# Autodesk Inventor assembly: craft
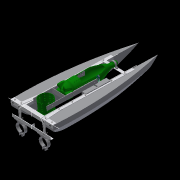
[picture p0: Inventor's stored thumbnail of the model, 180x180]
Saved by Autodesk Inventor 2016 (Build 200138000, 138)
## iProperties
Created: 2019-02-12
Part Number: craft
Document SubType Name: Assembly
Designer: Calb3e
Author: Calb3e
## Documents named in this file (24)
- C:\Users\Calb3\Documents\Inventor\water proj\craft.iam
- C:\Users\Calb3\Documents\Inventor\water proj\GeneralCraftShape4 (1).ipt
- C:\Users\Calb3\Documents\Inventor\water proj\Water Bottle.ipt
- C:\Users\Calb3\Documents\Inventor\water proj\Lbarx2.ipt
- C:\Users\Calb3\Documents\Inventor\water proj\half bottle.ipt
- C:\Users\Calb3\Documents\Inventor\water proj\Lbarx1 big.ipt
- C:\Users\Calb3\Documents\Inventor\water proj\flat bar1.ipt
- C:\Users\Calb3\Documents\Inventor\water proj\holder.ipt
- C:\Users\Calb3\Documents\Inventor\water proj\flatbarx2.ipt
- C:\Users\Calb3\Documents\Inventor\water proj\Lbarx1 small.ipt
- C:\Users\Calb3\Documents\Inventor\water proj\cushion.ipt
- C:\Users\Calb3\Documents\Inventor\water proj\pumpholder (1).ipt
- C:\Users\Calb3\Documents\Inventor\Content Center Files\R2016\en-US\ISO 7089\ISO 7089 - 5 - 140 HV(1).ipt
- C:\Users\Calb3\Documents\Inventor\Content Center Files\R2016\en-US\ISO 4762(2)\ISO 4762 - M5 x 20ISO.ipt
- C:\Users\Calb3\Documents\Inventor\Content Center Files\R2016\en-US\ISO 4032(2)\ISO 4032 - M5 - ISO.ipt
- C:\Users\Calb3\Documents\Inventor\Content Center Files\R2016\en-US\Wood screw 4 GOST 1145-80\Wood screw 4-5x22 GOST 1145-80.ipt
- C:\Users\Calb3\Documents\Inventor\Content Center Files\R2016\en-US\Screw GB_T 951-1986\Screw GB_T 951-1986 5 x 30.ipt
- C:\Users\Calb3\Documents\Inventor\water proj\extension.ipt
- C:\Users\Calb3\Documents\Inventor\water proj\extension2.ipt
- C:\Users\Calb3\Documents\Inventor\water proj\extension3.ipt
- C:\Users\Calb3\Documents\Inventor\water proj\support.ipt
- C:\Users\Calb3\Documents\Inventor\Content Center Files\R2016\en-US\ISO 4762(2)\ISO 4762 - M3 x 30ISO.ipt
- C:\Users\Calb3\Documents\Inventor\Content Center Files\R2016\en-US\ISO 4032(2)\ISO 4032 - M3 - ISO.ipt
- C:\Users\Calb3\Documents\Inventor\water proj\lastflat bar.ipt
## Components (88 placed, 23 different names)
1. GeneralCraftShape4 (1):1 — Mate:1, Mate:2, Mate:3, Mate:4, Mate:6, Angle:1
2. Lbarx2:1 — Mate:3, Mate:4, Mate:7, Insert:1, Mate:9, Mate:10, Mate:11, Mate:12, Insert:33, Insert:34, Insert:35, Insert:36
3. Lbarx2:2 — Mate:1, Mate:2, Insert:2, Mate:13, Mate:14, Mate:15, Mate:16, Insert:27, Insert:28, Insert:30, Insert:31, Insert:82
4. Water Bottle:1 — Insert:5, Angle:1
5. half bottle:1 — Mate:21
6. Lbarx1 big:1 — Mate:6, Mate:7, Insert:6, Insert:7, Insert:84
7. flat bar1:1 — Insert:1, Insert:2, Insert:3, Insert:4, Insert:29, Insert:32, Insert:50, Insert:51
8. holder:1 — Insert:3, Insert:4, Insert:5, Insert:38, Insert:39
9. flatbarx2:1 — Insert:7, Insert:9, Insert:23, Insert:24
10. flatbarx2:2 — Insert:6, Insert:8, Insert:19, Insert:20
11. Lbarx1 small:2 — Insert:8, Insert:9, Insert:10, Insert:11, Insert:12, Insert:13, Insert:21, Insert:22, Insert:42, Insert:43, Insert:44, Insert:45
12. cushion:1 — Mate:11, Mate:12
13. cushion:2 — Mate:13, Mate:14
14. cushion:3 — Mate:9, Mate:10
15. cushion:4 — Mate:15, Mate:16
16. pumpholder (1):1 — Insert:10, Insert:11, Insert:46, Insert:47
17. pumpholder (1):2 — Insert:12, Insert:13, Insert:48, Insert:49
18. ISO 7089 5 - 140 HV:1 — Insert:35, Insert:73
19. ISO 7089 5 - 140 HV:2 — Insert:32, Insert:70
20. ISO 7089 5 - 140 HV:3 — Insert:31, Insert:68
21. ISO 7089 5 - 140 HV:4 — Insert:30, Insert:67
22. ISO 7089 5 - 140 HV:5 — Insert:29, Insert:69
23. ISO 7089 5 - 140 HV:6 — Insert:28, Insert:66
24. ISO 7089 5 - 140 HV:12 — Insert:36, Insert:74
25. ISO 7089 5 - 140 HV:13 — Insert:34, Insert:72
26. ISO 7089 5 - 140 HV:14 — Insert:33, Insert:71
27. ISO 7089 5 - 140 HV:15 — Insert:59
28. ISO 7089 5 - 140 HV:18 — Insert:56
29. ISO 7089 5 - 140 HV:20 — Insert:22, Insert:62
30. ISO 7089 5 - 140 HV:21 — Insert:53
31. ISO 7089 5 - 140 HV:22 — Insert:19, Insert:52
32. ISO 7089 5 - 140 HV:23 — Insert:24, Insert:54
33. ISO 7089 5 - 140 HV:24 — Insert:23, Insert:61
34. ISO 7089 5 - 140 HV:25 — Insert:27, Insert:65
35. ISO 7089 5 - 140 HV:27 — Insert:55
36. ISO 7089 5 - 140 HV:28 — Insert:20, Insert:64
37. ISO 7089 5 - 140 HV:29 — Insert:21, Insert:63
38. ISO 4762 M5 x 20:1 — Insert:41
39. ISO 4762 M5 x 20:2 — Insert:40
40. ISO 4762 M5 x 20:3 — Insert:44
41. ISO 4762 M5 x 20:4 — Insert:45
42. ISO 4762 M5 x 20:5 — Insert:43
43. ISO 4762 M5 x 20:6 — Insert:42
44. ISO 7089 5 - 140 HV:30 — Insert:39, Insert:41
45. ISO 7089 5 - 140 HV:31 — Insert:38, Insert:40
46. ISO 4032 M5:1 — Insert:46
47. ISO 4032 M5:2 — Insert:47
48. ISO 4032 M5:3 — Insert:49
49. ISO 4032 M5:4 — Insert:48
50. ISO 4032 M5:5 — Insert:51
51. ISO 4032 M5:6 — Insert:50
52. Wood screw 4 GOST 1145-80 5x(22):1 — Insert:53
53. Wood screw 4 GOST 1145-80 5x(22):2 — Insert:55
54. Wood screw 4 GOST 1145-80 5x(22):3 — Insert:52
55. Wood screw 4 GOST 1145-80 5x(22):4 — Insert:54
56. Wood Screw GB/T 951-1986 M2.2 x 4.5-5-30:1 — Insert:61
57. Wood Screw GB/T 951-1986 M2.2 x 4.5-5-30:3 — Insert:62
58. Wood Screw GB/T 951-1986 M2.2 x 4.5-5-30:4 — Insert:63
59. Wood Screw GB/T 951-1986 M2.2 x 4.5-5-30:7 — Insert:56
60. Wood Screw GB/T 951-1986 M2.2 x 4.5-5-30:8 — Insert:59
61. Wood Screw GB/T 951-1986 M2.2 x 4.5-5-30:9 — Insert:64
62. Wood Screw GB/T 951-1986 M2.2 x 4.5-5-30:10 — Insert:65
63. Wood Screw GB/T 951-1986 M2.2 x 4.5-5-30:11 — Insert:66
64. Wood Screw GB/T 951-1986 M2.2 x 4.5-5-30:12 — Insert:68
65. Wood Screw GB/T 951-1986 M2.2 x 4.5-5-30:13 — Insert:67
66. Wood Screw GB/T 951-1986 M2.2 x 4.5-5-30:14 — Insert:69
67. Wood Screw GB/T 951-1986 M2.2 x 4.5-5-30:16 — Insert:74
68. Wood Screw GB/T 951-1986 M2.2 x 4.5-5-30:17 — Insert:73
69. Wood Screw GB/T 951-1986 M2.2 x 4.5-5-30:18 — Insert:72
70. Wood Screw GB/T 951-1986 M2.2 x 4.5-5-30:19 — Insert:71
71. Wood Screw GB/T 951-1986 M2.2 x 4.5-5-30:20 — Insert:70
72. extension:1 — Insert:76, Insert:77, Mate:18, Flush:2, Mate:19
73. extension2:1 — Insert:78, Insert:79, Mate:17, Flush:1, Mate:20, Mate:21, Insert:80
74. extension3:1 — Insert:78, Insert:79
75. extension3:2 — Insert:76, Insert:77
76. support:1 — Mate:17, Flush:1, Mate:18, Flush:2, Mate:19, Mate:20
77. ISO 4762 M3 x 30:1 — Insert:80, Mate:22, Flush:3
78. ISO 4032 M3:1 — Mate:22, Flush:3
79. lastflat bar:1 — Insert:82, Insert:87, Insert:88
80. lastflat bar:2 — Insert:84, Insert:85, Insert:86
81. Wood Screw GB/T 951-1986 M2.2 x 4.5-5-30:21 — Insert:92
82. Wood Screw GB/T 951-1986 M2.2 x 4.5-5-30:22 — Insert:89
83. Wood Screw GB/T 951-1986 M2.2 x 4.5-5-30:23 — Insert:91
84. Wood Screw GB/T 951-1986 M2.2 x 4.5-5-30:24 — Insert:90
85. ISO 7089 5 - 140 HV:32 — Insert:87, Insert:92
86. ISO 7089 5 - 140 HV:33 — Insert:86, Insert:91
87. ISO 7089 5 - 140 HV:34 — Insert:85, Insert:90
88. ISO 7089 5 - 140 HV:35 — Insert:88, Insert:89
## Relationships (102: Insert 78, Mate 20, Flush 3, Angle 1)
- Mate:1: GeneralCraftShape4 (1):1 ↔ Lbarx2:2
- Mate:2: GeneralCraftShape4 (1):1 ↔ Lbarx2:2
- Mate:3: GeneralCraftShape4 (1):1 ↔ Lbarx2:1
- Mate:4: GeneralCraftShape4 (1):1 ↔ Lbarx2:1
- Mate:6: GeneralCraftShape4 (1):1 ↔ Lbarx1 big:1
- Mate:7: Lbarx2:1 ↔ Lbarx1 big:1
- Insert:1: Lbarx2:1 ↔ flat bar1:1
- Insert:2: Lbarx2:2 ↔ flat bar1:1
- Insert:3: flat bar1:1 ↔ holder:1
- Insert:4: flat bar1:1 ↔ holder:1
- Insert:5: Water Bottle:1 ↔ holder:1
- Angle:1 (90 deg): GeneralCraftShape4 (1):1 ↔ Water Bottle:1
- Insert:6: Lbarx1 big:1 ↔ flatbarx2:2
- Insert:7: Lbarx1 big:1 ↔ flatbarx2:1
- Insert:8: flatbarx2:2 ↔ Lbarx1 small:2
- Insert:9: flatbarx2:1 ↔ Lbarx1 small:2
- Mate:9: Lbarx2:1 ↔ cushion:3
- Mate:10: Lbarx2:1 ↔ cushion:3
- Mate:11: Lbarx2:1 ↔ cushion:1
- Mate:12: Lbarx2:1 ↔ cushion:1
- Mate:13: Lbarx2:2 ↔ cushion:2
- Mate:14: Lbarx2:2 ↔ cushion:2
- Mate:15: Lbarx2:2 ↔ cushion:4
- Mate:16: Lbarx2:2 ↔ cushion:4
- Insert:10: Lbarx1 small:2 ↔ pumpholder (1):1
- Insert:11: Lbarx1 small:2 ↔ pumpholder (1):1
- Insert:12: Lbarx1 small:2 ↔ pumpholder (1):2
- Insert:13: Lbarx1 small:2 ↔ pumpholder (1):2
- Insert:19: flatbarx2:2 ↔ ISO 7089 5 - 140 HV:22
- Insert:20: flatbarx2:2 ↔ ISO 7089 5 - 140 HV:28
- Insert:21: Lbarx1 small:2 ↔ ISO 7089 5 - 140 HV:29
- Insert:22: Lbarx1 small:2 ↔ ISO 7089 5 - 140 HV:20
- Insert:23: flatbarx2:1 ↔ ISO 7089 5 - 140 HV:24
- Insert:24: flatbarx2:1 ↔ ISO 7089 5 - 140 HV:23
- Insert:27: Lbarx2:2 ↔ ISO 7089 5 - 140 HV:25
- Insert:28: Lbarx2:2 ↔ ISO 7089 5 - 140 HV:6
- Insert:29: flat bar1:1 ↔ ISO 7089 5 - 140 HV:5
- Insert:30: Lbarx2:2 ↔ ISO 7089 5 - 140 HV:4
- Insert:31: Lbarx2:2 ↔ ISO 7089 5 - 140 HV:3
- Insert:32: flat bar1:1 ↔ ISO 7089 5 - 140 HV:2
- Insert:33: Lbarx2:1 ↔ ISO 7089 5 - 140 HV:14
- Insert:34: Lbarx2:1 ↔ ISO 7089 5 - 140 HV:13
- Insert:35: Lbarx2:1 ↔ ISO 7089 5 - 140 HV:1
- Insert:36: Lbarx2:1 ↔ ISO 7089 5 - 140 HV:12
- Insert:38: holder:1 ↔ ISO 7089 5 - 140 HV:31
- Insert:39: holder:1 ↔ ISO 7089 5 - 140 HV:30
- Insert:40: ISO 4762 M5 x 20:2 ↔ ISO 7089 5 - 140 HV:31
- Insert:41: ISO 4762 M5 x 20:1 ↔ ISO 7089 5 - 140 HV:30
- Insert:42: Lbarx1 small:2 ↔ ISO 4762 M5 x 20:6
- Insert:43: Lbarx1 small:2 ↔ ISO 4762 M5 x 20:5
- Insert:44: Lbarx1 small:2 ↔ ISO 4762 M5 x 20:3
- Insert:45: Lbarx1 small:2 ↔ ISO 4762 M5 x 20:4
- Insert:46: pumpholder (1):1 ↔ ISO 4032 M5:1
- Insert:47: pumpholder (1):1 ↔ ISO 4032 M5:2
- Insert:48: pumpholder (1):2 ↔ ISO 4032 M5:4
- Insert:49: pumpholder (1):2 ↔ ISO 4032 M5:3
- Insert:50: flat bar1:1 ↔ ISO 4032 M5:6
- Insert:51: flat bar1:1 ↔ ISO 4032 M5:5
- Insert:52: ISO 7089 5 - 140 HV:22 ↔ Wood screw 4 GOST 1145-80 5x(22):3
- Insert:53: ISO 7089 5 - 140 HV:21 ↔ Wood screw 4 GOST 1145-80 5x(22):1
- Insert:54: ISO 7089 5 - 140 HV:23 ↔ Wood screw 4 GOST 1145-80 5x(22):4
- Insert:55: ISO 7089 5 - 140 HV:27 ↔ Wood screw 4 GOST 1145-80 5x(22):2
- Insert:56: ISO 7089 5 - 140 HV:18 ↔ Wood Screw GB/T 951-1986 M2.2 x 4.5-5-30:7
- Insert:59: ISO 7089 5 - 140 HV:15 ↔ Wood Screw GB/T 951-1986 M2.2 x 4.5-5-30:8
- Insert:61: ISO 7089 5 - 140 HV:24 ↔ Wood Screw GB/T 951-1986 M2.2 x 4.5-5-30:1
- Insert:62: ISO 7089 5 - 140 HV:20 ↔ Wood Screw GB/T 951-1986 M2.2 x 4.5-5-30:3
- Insert:63: ISO 7089 5 - 140 HV:29 ↔ Wood Screw GB/T 951-1986 M2.2 x 4.5-5-30:4
- Insert:64: ISO 7089 5 - 140 HV:28 ↔ Wood Screw GB/T 951-1986 M2.2 x 4.5-5-30:9
- Insert:65: ISO 7089 5 - 140 HV:25 ↔ Wood Screw GB/T 951-1986 M2.2 x 4.5-5-30:10
- Insert:66: ISO 7089 5 - 140 HV:6 ↔ Wood Screw GB/T 951-1986 M2.2 x 4.5-5-30:11
- Insert:67: ISO 7089 5 - 140 HV:4 ↔ Wood Screw GB/T 951-1986 M2.2 x 4.5-5-30:13
- Insert:68: ISO 7089 5 - 140 HV:3 ↔ Wood Screw GB/T 951-1986 M2.2 x 4.5-5-30:12
- Insert:69: ISO 7089 5 - 140 HV:5 ↔ Wood Screw GB/T 951-1986 M2.2 x 4.5-5-30:14
- Insert:70: ISO 7089 5 - 140 HV:2 ↔ Wood Screw GB/T 951-1986 M2.2 x 4.5-5-30:20
- Insert:71: ISO 7089 5 - 140 HV:14 ↔ Wood Screw GB/T 951-1986 M2.2 x 4.5-5-30:19
- Insert:72: ISO 7089 5 - 140 HV:13 ↔ Wood Screw GB/T 951-1986 M2.2 x 4.5-5-30:18
- Insert:73: ISO 7089 5 - 140 HV:1 ↔ Wood Screw GB/T 951-1986 M2.2 x 4.5-5-30:17
- Insert:74: ISO 7089 5 - 140 HV:12 ↔ Wood Screw GB/T 951-1986 M2.2 x 4.5-5-30:16
- Insert:76: extension:1 ↔ extension3:2
- Insert:77: extension:1 ↔ extension3:2
- Insert:78: extension2:1 ↔ extension3:1
- Insert:79: extension2:1 ↔ extension3:1
- Mate:17: extension2:1 ↔ support:1
- Flush:1: extension2:1 ↔ support:1
- Mate:18: extension:1 ↔ support:1
- Flush:2: extension:1 ↔ support:1
- Mate:19: extension:1 ↔ support:1
- Mate:20: extension2:1 ↔ support:1
- Mate:21: half bottle:1 ↔ extension2:1
- Insert:80: extension2:1 ↔ ISO 4762 M3 x 30:1
- Mate:22: ISO 4762 M3 x 30:1 ↔ ISO 4032 M3:1
- Flush:3: ISO 4762 M3 x 30:1 ↔ ISO 4032 M3:1
- Insert:82: Lbarx2:2 ↔ lastflat bar:1
- Insert:84: Lbarx1 big:1 ↔ lastflat bar:2
- Insert:85: lastflat bar:2 ↔ ISO 7089 5 - 140 HV:34
- Insert:86: lastflat bar:2 ↔ ISO 7089 5 - 140 HV:33
- Insert:87: lastflat bar:1 ↔ ISO 7089 5 - 140 HV:32
- Insert:88: lastflat bar:1 ↔ ISO 7089 5 - 140 HV:35
- Insert:89: Wood Screw GB/T 951-1986 M2.2 x 4.5-5-30:22 ↔ ISO 7089 5 - 140 HV:35
- Insert:90: Wood Screw GB/T 951-1986 M2.2 x 4.5-5-30:24 ↔ ISO 7089 5 - 140 HV:34
- Insert:91: Wood Screw GB/T 951-1986 M2.2 x 4.5-5-30:23 ↔ ISO 7089 5 - 140 HV:33
- Insert:92: Wood Screw GB/T 951-1986 M2.2 x 4.5-5-30:21 ↔ ISO 7089 5 - 140 HV:32
